# Autodesk Inventor assembly: delorean 1
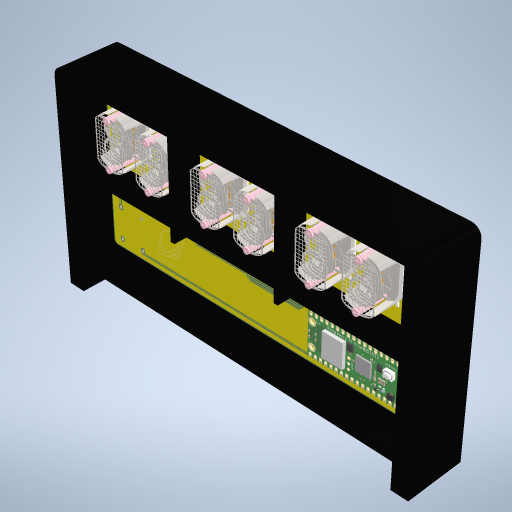
[picture p0: Inventor's stored thumbnail of the model, 512x512]
Saved by Autodesk Inventor 2024.3 (Build 283343000, 343)
## iProperties
Company: Kicad
Created: 2025-06-10
Part Number: delorean 1
Description: KiCad electronic assembly
Document SubType Name: Assembly
Designer: megha
Authority: Unknown
Sending System: KiCad to STEP converter
Preprocessor: Open CASCADE STEP processor 7.8
Title: delorean.step
Author: Pcbnew
## Documents named in this file (14)
- C:\Users\megha\KiCad\8.99\projects\delorean\CAD\board\delorean.iam
- C:\Users\megha\KiCad\8.99\projects\delorean\CAD\board\DIP16.ipt
- C:\Users\megha\KiCad\8.99\projects\delorean\CAD\board\R_0805_2012Metric.ipt
- C:\Users\megha\KiCad\8.99\projects\delorean\CAD\board\IN-12 Nixie Tube.iam
- C:\Users\megha\KiCad\8.99\projects\delorean\CAD\board\RaspberryPi Pico W v2.iam
- C:\Users\megha\KiCad\8.99\projects\delorean\CAD\board\delorean_copper.ipt
- C:\Users\megha\KiCad\8.99\projects\delorean\CAD\board\delorean_pad.ipt
- C:\Users\megha\KiCad\8.99\projects\delorean\CAD\board\delorean_via.ipt
- C:\Users\megha\KiCad\8.99\projects\delorean\CAD\board\delorean_silkscreen.ipt
- C:\Users\megha\KiCad\8.99\projects\delorean\CAD\board\delorean_PCB.ipt
- C:\Users\megha\KiCad\8.99\projects\delorean\CAD\case\case.ipt
- C:\Users\megha\KiCad\8.99\projects\delorean\CAD\acrylicDoor.ipt
- C:\Users\megha\KiCad\8.99\projects\delorean\CAD\HL050-2\HL050-2\HL050-2\HL050-2.iam
- C:\Users\megha\KiCad\8.99\projects\delorean\CAD\HL050-2\HL050-2\HL050-2\HINGE-HENGZHU-40X40-A1.ipt
## Components (28 placed, 28 different names)
1. case:1 — Mate:3
2. HINGE-HENGZHU-40X40-A1_2 — Mate:4, Mate:5, Mate:6, Mate:7
3. acrylicDoor:1 — Mate:6, Mate:7
4. HL050-2:1 [sub-assembly] — Mate:3, Mate:4, Mate:5
5. 1
6. 2
7. 3
8. 4
9. 56 [sub-assembly]
10. 57
11. 58
12. 59
13. 60
14. 61 [sub-assembly]
15. 62
16. 142 [sub-assembly]
17. 143
18. 144
19. 145 [sub-assembly]
20. 146 [sub-assembly]
21. 147 [sub-assembly]
22. 148 [sub-assembly]
23. 149
24. 150
25. 151
26. 152
27. 153
28. 154
## Relationships (5: Mate 5)
- Mate:3: case:1 ↔ HL050-2:1
- Mate:4: HINGE-HENGZHU-40X40-A1_2 ↔ HL050-2:1
- Mate:5: HINGE-HENGZHU-40X40-A1_2 ↔ HL050-2:1
- Mate:6: HINGE-HENGZHU-40X40-A1_2 ↔ acrylicDoor:1
- Mate:7: HINGE-HENGZHU-40X40-A1_2 ↔ acrylicDoor:1
